# Autodesk Inventor assembly: Pressure Vessel, Global Assembly
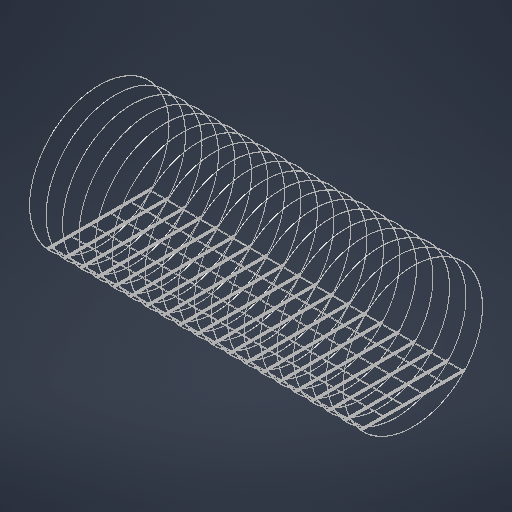
[picture p0: Inventor's stored thumbnail of the model, 512x512]
Saved by Autodesk Inventor 2026 (Build 300175000, 175)
## iProperties
Created: 2025-10-25
Part Number: Pressure Vessel, Global Assembly
Document SubType Name: Assembly
Designer: Brandon Portillo
Author: Brandon Portillo
## Documents named in this file (6)
- C:\Users\anarc\GitHub\TSGC-NASA_Senior_Design\CAD\Pressure Vessel\Pressure Vessel, Global Assembly.iam
- C:\Users\anarc\GitHub\TSGC-NASA_Senior_Design\CAD\Pressure Vessel\Pressure Vessel, Single Part.ipt
- C:\Users\anarc\GitHub\TSGC-NASA_Senior_Design\CAD\Pressure Vessel\Floor, Uncutt.ipt
- C:\Users\anarc\GitHub\TSGC-NASA_Senior_Design\CAD\Pressure Vessel\Support Ring.ipt
- C:\Users\anarc\GitHub\TSGC-NASA_Senior_Design\CAD\Pressure Vessel\Floor Frame.ipt
- C:\Users\anarc\GitHub\TSGC-NASA_Senior_Design\CAD\Pressure Vessel\FLoor Frame, Small.ipt
## Components (156 placed, 5 different names)
1. Pressure Vessel, Single Part:1 — Flush:7, Tangent:3, Tangent:4, Tangent:5, Mate:7, Flush:14
2. Floor, Uncutt:1 — Flush:7, Tangent:3, Tangent:4, Angle:1, Mate:4, Mate:6, Flush:13
3. Support Ring:3 — Mate:3, Mate:7, Flush:14
4. Support Ring:4
5. Support Ring:5
6. Support Ring:6
7. Support Ring:7
8. Support Ring:8
9. Support Ring:9
10. Support Ring:10
11. Support Ring:11
12. Support Ring:12
13. Support Ring:13
14. Support Ring:14
15. Support Ring:15
16. Support Ring:16
17. Support Ring:17
18. Support Ring:18
19. Support Ring:19
20. Support Ring:20
21. Support Ring:21
22. Support Ring:22
23. Floor Frame:1 — Mate:3, Mate:4, Tangent:5, Mate:5
24. Floor Frame:2
25. Floor Frame:3
26. Floor Frame:4
27. Floor Frame:5
28. Floor Frame:6
29. Floor Frame:7
30. Floor Frame:8
31. Floor Frame:9
32. Floor Frame:10
33. Floor Frame:11
34. Floor Frame:12
35. Floor Frame:13
36. Floor Frame:14
37. Floor Frame:15
38. Floor Frame:16
39. Floor Frame:17
40. Floor Frame:18
41. Floor Frame:19
42. Floor Frame:20
43. FLoor Frame, Small:1 — Mate:5, Mate:6, Flush:13
44. FLoor Frame, Small:2
45. FLoor Frame, Small:3
46. FLoor Frame, Small:4
47. FLoor Frame, Small:5
48. FLoor Frame, Small:6
49. FLoor Frame, Small:7
50. FLoor Frame, Small:8
51. FLoor Frame, Small:9
52. FLoor Frame, Small:10
53. FLoor Frame, Small:11
54. FLoor Frame, Small:12
55. FLoor Frame, Small:13
56. FLoor Frame, Small:14
57. FLoor Frame, Small:15
58. FLoor Frame, Small:16
59. FLoor Frame, Small:17
60. FLoor Frame, Small:18
61. FLoor Frame, Small:19
62. FLoor Frame, Small:21
63. FLoor Frame, Small:22
64. FLoor Frame, Small:23
65. FLoor Frame, Small:24
66. FLoor Frame, Small:25
67. FLoor Frame, Small:26
68. FLoor Frame, Small:27
69. FLoor Frame, Small:28
70. FLoor Frame, Small:29
71. FLoor Frame, Small:30
72. FLoor Frame, Small:31
73. FLoor Frame, Small:32
74. FLoor Frame, Small:33
75. FLoor Frame, Small:34
76. FLoor Frame, Small:35
77. FLoor Frame, Small:36
78. FLoor Frame, Small:37
79. FLoor Frame, Small:38
80. FLoor Frame, Small:39
81. FLoor Frame, Small:41
82. FLoor Frame, Small:42
83. FLoor Frame, Small:43
84. FLoor Frame, Small:44
85. FLoor Frame, Small:45
86. FLoor Frame, Small:46
87. FLoor Frame, Small:47
88. FLoor Frame, Small:48
89. FLoor Frame, Small:49
90. FLoor Frame, Small:50
91. FLoor Frame, Small:51
92. FLoor Frame, Small:52
93. FLoor Frame, Small:53
94. FLoor Frame, Small:54
95. FLoor Frame, Small:55
96. FLoor Frame, Small:56
97. FLoor Frame, Small:57
98. FLoor Frame, Small:58
99. FLoor Frame, Small:59
100. FLoor Frame, Small:61
101. FLoor Frame, Small:62
102. FLoor Frame, Small:63
103. FLoor Frame, Small:64
104. FLoor Frame, Small:65
105. FLoor Frame, Small:66
106. FLoor Frame, Small:67
107. FLoor Frame, Small:68
108. FLoor Frame, Small:69
109. FLoor Frame, Small:70
110. FLoor Frame, Small:71
111. FLoor Frame, Small:72
112. FLoor Frame, Small:73
113. FLoor Frame, Small:74
114. FLoor Frame, Small:75
115. FLoor Frame, Small:76
116. FLoor Frame, Small:77
117. FLoor Frame, Small:78
118. FLoor Frame, Small:79
119. FLoor Frame, Small:81
120. FLoor Frame, Small:82
121. FLoor Frame, Small:83
122. FLoor Frame, Small:84
123. FLoor Frame, Small:85
124. FLoor Frame, Small:86
125. FLoor Frame, Small:87
126. FLoor Frame, Small:88
127. FLoor Frame, Small:89
128. FLoor Frame, Small:90
129. FLoor Frame, Small:91
130. FLoor Frame, Small:92
131. FLoor Frame, Small:93
132. FLoor Frame, Small:94
133. FLoor Frame, Small:95
134. FLoor Frame, Small:96
135. FLoor Frame, Small:97
136. FLoor Frame, Small:98
137. FLoor Frame, Small:99
138. FLoor Frame, Small:101
139. FLoor Frame, Small:102
140. FLoor Frame, Small:103
141. FLoor Frame, Small:104
142. FLoor Frame, Small:105
143. FLoor Frame, Small:106
144. FLoor Frame, Small:107
145. FLoor Frame, Small:108
146. FLoor Frame, Small:109
147. FLoor Frame, Small:110
148. FLoor Frame, Small:111
149. FLoor Frame, Small:112
150. FLoor Frame, Small:113
151. FLoor Frame, Small:114
152. FLoor Frame, Small:115
153. FLoor Frame, Small:116
154. FLoor Frame, Small:117
155. FLoor Frame, Small:118
156. FLoor Frame, Small:119
## Component patterns: (20 elements, first: Support Ring:3), (20 elements, first: Floor Frame:1), (114 elements, first: FLoor Frame, Small:1)
## Relationships (12: Mate 5, Flush 3, Tangent 3, Angle 1)
- Flush:7: Pressure Vessel, Single Part:1 ↔ Floor, Uncutt:1
- Tangent:3: Pressure Vessel, Single Part:1 ↔ Floor, Uncutt:1
- Tangent:4: Pressure Vessel, Single Part:1 ↔ Floor, Uncutt:1
- Angle:1 (0 deg): Floor, Uncutt:1
- Mate:3: Support Ring:3 ↔ Floor Frame:1
- Mate:4: Floor, Uncutt:1 ↔ Floor Frame:1
- Tangent:5: Pressure Vessel, Single Part:1 ↔ Floor Frame:1
- Mate:5: Floor Frame:1 ↔ FLoor Frame, Small:1
- Mate:6: Floor, Uncutt:1 ↔ FLoor Frame, Small:1
- Flush:13 (125 mm): Floor, Uncutt:1 ↔ FLoor Frame, Small:1
- Mate:7: Pressure Vessel, Single Part:1 ↔ Support Ring:3
- Flush:14 (250 mm): Pressure Vessel, Single Part:1 ↔ Support Ring:3
